# Autodesk Inventor assembly: test assembly
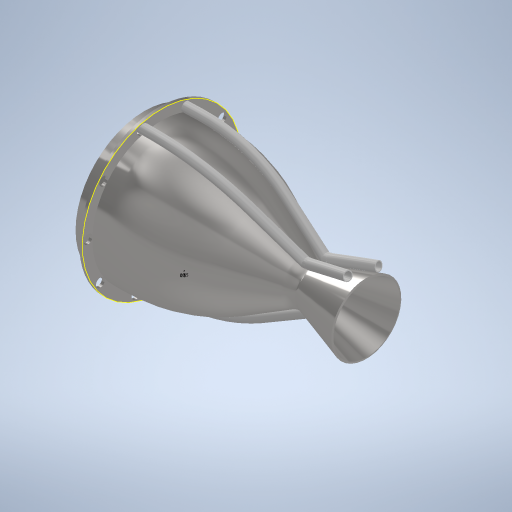
[picture p0: Inventor's stored thumbnail of the model, 512x512]
Saved by Autodesk Inventor 2023 (Build 270158000, 158)
## iProperties
Created: 2022-07-21
Part Number: test assembly
Document SubType Name: Assembly
Designer: station
Author: station
## Documents named in this file (7)
- C:\Users\station\Documents\Project\Liquid-engine-cooling-system\liquid_engine_design\Ethanol engine 5 -inventor\test assembly.iam
- C:\Users\station\Documents\Project\Liquid-engine-cooling-system\liquid_engine_design\Ethanol engine 5 -inventor\inner wall.ipt
- C:\Users\station\Documents\Project\Liquid-engine-cooling-system\liquid_engine_design\Ethanol engine 5 -inventor\new outer wall.ipt
- C:\Users\station\Documents\Project\Liquid-engine-cooling-system\liquid_engine_design\Ethanol engine 5 -inventor\back bracket 2.ipt
- C:\Users\station\Documents\Project\Liquid-engine-cooling-system\liquid_engine_design\Ethanol engine 5 -inventor\back bracket.ipt
- C:\Users\station\Documents\Project\Liquid-engine-cooling-system\liquid_engine_design\Ethanol engine 5 -inventor\bracket 1.ipt
- C:\Users\station\Documents\Project\Liquid-engine-cooling-system\liquid_engine_design\Ethanol engine 5 -inventor\ethanol engine 5 v7.iam
## Components (8 placed, 6 different names)
1. inner wall:1 — Mate:1, Flush:1, Mate:2, Mate:4, Tangent:1, Tangent:2, Tangent:3, Tangent:4, Tangent:5, Tangent:6
2. new outer wall:1 — Mate:1, Flush:1, Mate:3, Mate:5, Mate:6, Mate:7
3. back bracket 2:1 — Mate:2, Mate:3, Mate:8
4. back bracket:1 — Mate:4, Mate:5, Mate:8, Mate:9
5. bracket 1:1 — Mate:6, Mate:7, Mate:9
6. ethanol engine 5 v7:1 [sub-assembly] — Tangent:1, Tangent:2
7. ethanol engine 5 v7:2 [sub-assembly] — Tangent:3, Tangent:4
8. ethanol engine 5 v7:3 [sub-assembly] — Tangent:5, Tangent:6
## Relationships (16: Mate 9, Tangent 6, Flush 1)
- Mate:1: inner wall:1 ↔ new outer wall:1
- Flush:1: inner wall:1 ↔ new outer wall:1
- Mate:2: inner wall:1 ↔ back bracket 2:1
- Mate:3 (-14.601 mm): new outer wall:1 ↔ back bracket 2:1
- Mate:4: inner wall:1 ↔ back bracket:1
- Mate:5 (-3.601 mm): new outer wall:1 ↔ back bracket:1
- Mate:6: new outer wall:1 ↔ bracket 1:1
- Mate:7 (-18 mm): new outer wall:1 ↔ bracket 1:1
- Mate:8: back bracket 2:1 ↔ back bracket:1
- Mate:9: back bracket:1 ↔ bracket 1:1
- Tangent:1: inner wall:1 ↔ ethanol engine 5 v7:1
- Tangent:2: inner wall:1 ↔ ethanol engine 5 v7:1
- Tangent:3: inner wall:1 ↔ ethanol engine 5 v7:2
- Tangent:4: inner wall:1 ↔ ethanol engine 5 v7:2
- Tangent:5: inner wall:1 ↔ ethanol engine 5 v7:3
- Tangent:6: inner wall:1 ↔ ethanol engine 5 v7:3
